# Autodesk Inventor assembly: STAGE1,ELEVATOR
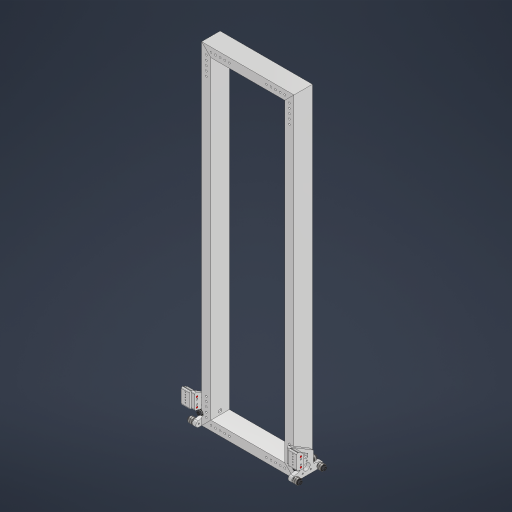
[picture p0: Inventor's stored thumbnail of the model, 512x512]
Saved by Autodesk Inventor 2024.3 (Build 283343010, 343A)
## iProperties
ILogicPurgeVersion: 0.0.0.0
OnSaveVersion: 3.4.3.0
OnSaveAssembly: COREAutomationManager
Created: 2025-02-04
Part Number: STAGE1,ELEVATOR
Document SubType Name: Assembly
Designer: Jthib
Mfg Approved By: John.Thibert
Mass: 3379.46 g
Surface Area: 7569.45 cm^2
Volume: 1217.87 cm^3
Density: 2.7749 g/cm^3
ModelCat: Uncategorized
CN_MASS: 3.38
Author: Jthib
## Documents named in this file (8)
- C:\Users\Owen\Documents\GitHub\2025-Poseidon-Mechanical\STAGE1,ELEVATOR.iam
- C:\Users\Owen\Documents\GitHub\2025-Poseidon-Mechanical\TUBE,ELEVATOR,SIDE,STAGE1.ipt
- C:\Users\Owen\Documents\GitHub\2025-Poseidon-Mechanical\TUBE,ELEVATOR,BOT,STAGE1.ipt
- C:\Users\Owen\Documents\GitHub\2025-Poseidon-Mechanical\PLATE,BRACKET,ELEVATOR,STAGE1.ipt
- C:\Users\Owen\Documents\GitHub\2025-Poseidon-Mechanical\TUBE,ELEVATOR,TOP,STAGE1.ipt
- C:\Users\Owen\Documents\GitHub\2025-Poseidon-Mechanical\SLIDE,ELEVATOR,STAGE1,LH.iam
- C:\Users\Owen\Documents\GitHub\2025-Poseidon-Mechanical\SLIDE,ELEVATOR,STAGE1,RH.iam
- C:\Users\Owen\Documents\GitHub\2025-Poseidon-Mechanical\BRACE,CHAIN,#25,ELEVATOR.ipt
## Components (16 placed, 7 different names)
1. SLIDE,ELEVATOR,STAGE1,LH.iam:1 [sub-assembly] — Mate:15
2. SLIDE,ELEVATOR,STAGE1,RH.iam:1 [sub-assembly]
3. TUBE,ELEVATOR,TOP,STAGE1.ipt:1
4. TUBE,ELEVATOR,BOT,STAGE1.ipt:1 — Mate:14
5. TUBE,ELEVATOR,SIDE,STAGE1.ipt:1 — Mate:13, Symmetry:1
6. TUBE,ELEVATOR,SIDE,STAGE1.ipt:2 — Symmetry:1
7. BRACE,CHAIN,#25,ELEVATOR.ipt:1
8. BRACE,CHAIN,#25,ELEVATOR.ipt:2
9. PLATE,BRACKET,ELEVATOR,STAGE1.ipt:1
10. PLATE,BRACKET,ELEVATOR,STAGE1.ipt:2
11. PLATE,BRACKET,ELEVATOR,STAGE1.ipt:3
12. PLATE,BRACKET,ELEVATOR,STAGE1.ipt:4
13. PLATE,BRACKET,ELEVATOR,STAGE1.ipt:5
14. PLATE,BRACKET,ELEVATOR,STAGE1.ipt:6
15. PLATE,BRACKET,ELEVATOR,STAGE1.ipt:7
16. PLATE,BRACKET,ELEVATOR,STAGE1.ipt:8
## Component patterns: (2 elements, first: PLATE,BRACKET,ELEVATOR,STAGE1.ipt:1 + PLATE,BRACKET,ELEVATOR,STAGE1.ipt:2 + PLATE,BRACKET,ELEVATOR,STAGE1.ipt:3 + PLATE,BRACKET,ELEVATOR,STAGE1.ipt:4)
## Relationships (32: Insert 16, Mate 15, Symmetry 1)
- [Insert]: TUBE,ELEVATOR,BOT,STAGE1.ipt:1 ↔ PLATE,BRACKET,ELEVATOR,STAGE1.ipt:1
- [Insert]: TUBE,ELEVATOR,BOT,STAGE1.ipt:1 ↔ PLATE,BRACKET,ELEVATOR,STAGE1.ipt:1
- [Insert]: TUBE,ELEVATOR,BOT,STAGE1.ipt:1 ↔ PLATE,BRACKET,ELEVATOR,STAGE1.ipt:2
- [Insert]: TUBE,ELEVATOR,BOT,STAGE1.ipt:1 ↔ PLATE,BRACKET,ELEVATOR,STAGE1.ipt:2
- [Insert]: TUBE,ELEVATOR,SIDE,STAGE1.ipt:2 ↔ PLATE,BRACKET,ELEVATOR,STAGE1.ipt:2
- [Insert]: TUBE,ELEVATOR,SIDE,STAGE1.ipt:2 ↔ PLATE,BRACKET,ELEVATOR,STAGE1.ipt:2
- [Insert]: TUBE,ELEVATOR,TOP,STAGE1.ipt:1 ↔ PLATE,BRACKET,ELEVATOR,STAGE1.ipt:3
- [Insert]: TUBE,ELEVATOR,TOP,STAGE1.ipt:1 ↔ PLATE,BRACKET,ELEVATOR,STAGE1.ipt:3
- [Insert]: TUBE,ELEVATOR,TOP,STAGE1.ipt:1 ↔ PLATE,BRACKET,ELEVATOR,STAGE1.ipt:4
- [Insert]: TUBE,ELEVATOR,TOP,STAGE1.ipt:1 ↔ PLATE,BRACKET,ELEVATOR,STAGE1.ipt:4
- [Insert]: TUBE,ELEVATOR,SIDE,STAGE1.ipt:2 ↔ PLATE,BRACKET,ELEVATOR,STAGE1.ipt:4
- [Insert]: TUBE,ELEVATOR,SIDE,STAGE1.ipt:2 ↔ PLATE,BRACKET,ELEVATOR,STAGE1.ipt:4
- [Insert]: TUBE,ELEVATOR,SIDE,STAGE1.ipt:1 ↔ PLATE,BRACKET,ELEVATOR,STAGE1.ipt:1
- [Insert]: TUBE,ELEVATOR,SIDE,STAGE1.ipt:1 ↔ PLATE,BRACKET,ELEVATOR,STAGE1.ipt:1
- [Insert]: TUBE,ELEVATOR,SIDE,STAGE1.ipt:1 ↔ PLATE,BRACKET,ELEVATOR,STAGE1.ipt:3
- [Insert]: TUBE,ELEVATOR,SIDE,STAGE1.ipt:1 ↔ PLATE,BRACKET,ELEVATOR,STAGE1.ipt:3
- [Mate]: SLIDE,ELEVATOR,STAGE1,RH.iam:1 ↔ TUBE,ELEVATOR,SIDE,STAGE1.ipt:2
- [Mate]: SLIDE,ELEVATOR,STAGE1,RH.iam:1 ↔ TUBE,ELEVATOR,SIDE,STAGE1.ipt:2
- [Mate]: SLIDE,ELEVATOR,STAGE1,RH.iam:1 ↔ TUBE,ELEVATOR,SIDE,STAGE1.ipt:2
- [Mate]: SLIDE,ELEVATOR,STAGE1,LH.iam:1 ↔ TUBE,ELEVATOR,SIDE,STAGE1.ipt:1
- [Mate]: SLIDE,ELEVATOR,STAGE1,LH.iam:1 ↔ TUBE,ELEVATOR,SIDE,STAGE1.ipt:1
- [Mate]: SLIDE,ELEVATOR,STAGE1,LH.iam:1 ↔ TUBE,ELEVATOR,SIDE,STAGE1.ipt:1
- [Mate]: SLIDE,ELEVATOR,STAGE1,RH.iam:1 ↔ BRACE,CHAIN,#25,ELEVATOR.ipt:1
- [Mate]: SLIDE,ELEVATOR,STAGE1,RH.iam:1 ↔ BRACE,CHAIN,#25,ELEVATOR.ipt:1
- [Mate]: SLIDE,ELEVATOR,STAGE1,RH.iam:1 ↔ BRACE,CHAIN,#25,ELEVATOR.ipt:1
- [Mate]: SLIDE,ELEVATOR,STAGE1,LH.iam:1 ↔ BRACE,CHAIN,#25,ELEVATOR.ipt:2
- [Mate]: SLIDE,ELEVATOR,STAGE1,LH.iam:1 ↔ BRACE,CHAIN,#25,ELEVATOR.ipt:2
- [Mate]: SLIDE,ELEVATOR,STAGE1,LH.iam:1 ↔ BRACE,CHAIN,#25,ELEVATOR.ipt:2
- Mate:13 (-127 mm): TUBE,ELEVATOR,SIDE,STAGE1.ipt:1
- Mate:14 (-457.2 mm): TUBE,ELEVATOR,BOT,STAGE1.ipt:1
- Mate:15: SLIDE,ELEVATOR,STAGE1,LH.iam:1
- Symmetry:1: TUBE,ELEVATOR,SIDE,STAGE1.ipt:1 ↔ TUBE,ELEVATOR,SIDE,STAGE1.ipt:2
